# Autodesk Inventor assembly: wheel-assembly
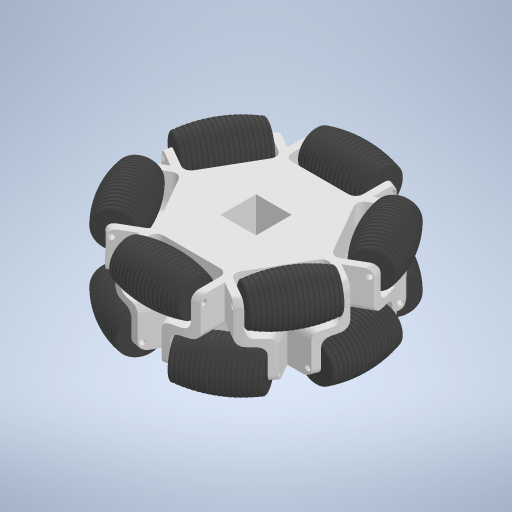
[picture p0: Inventor's stored thumbnail of the model, 512x512]
Saved by Autodesk Inventor 2024.2 (Build 282272000, 272)
## iProperties
Created: 2024-04-23
Part Number: wheel-assembly
Document SubType Name: Assembly
Designer: Robin
Author: Robin
## Documents named in this file (3)
- C:\Users\Robin\Desktop\CAD\wheel-assembly.iam
- C:\Users\Robin\Desktop\CAD\holo-5-wheel.ipt
- C:\Users\Robin\Desktop\CAD\roller-5.ipt
## Components (13 placed, 2 different names)
1. holo-5-wheel:1 — Mate:1, Mate:2, Mate:3, Mate:4
2. roller-5:1 — Mate:1, Mate:2
3. roller-5:2
4. roller-5:3
5. roller-5:4
6. roller-5:5
7. roller-5:6
8. roller-5:7 — Mate:3, Mate:4
9. roller-5:8
10. roller-5:9
11. roller-5:10
12. roller-5:11
13. roller-5:12
## Component patterns: (6 elements, first: roller-5:1), (6 elements, first: roller-5:7)
## Relationships (4: Mate 4)
- Mate:1: holo-5-wheel:1 ↔ roller-5:1
- Mate:2 (0.25 mm): holo-5-wheel:1 ↔ roller-5:1
- Mate:3 (0.25 mm): holo-5-wheel:1 ↔ roller-5:7
- Mate:4: holo-5-wheel:1 ↔ roller-5:7
